# Autodesk Inventor assembly: sub assembly 2iam
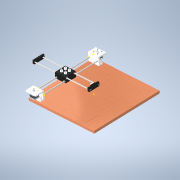
[picture p0: Inventor's stored thumbnail of the model, 180x180]
Saved by Autodesk Inventor 2021 (Build 250183000, 183)
## iProperties
Created: 2021-07-13
Part Number: sub assembly 2iam
Document SubType Name: Assembly
Designer: Michael Swaminathan
Author: Michael Swaminathan
## Documents named in this file (9)
- F:\Pattern Drawing Bot\Xy plotter Drawing Machine\sub assembly 2iam.iam
- F:\Pattern Drawing Bot\Xy plotter Drawing Machine\base.ipt
- F:\Pattern Drawing Bot\Xy plotter Drawing Machine\Motor With Support Assembly.iam
- F:\Pattern Drawing Bot\Xy plotter Drawing Machine\Guidance Rods 2.ipt
- F:\Pattern Drawing Bot\Xy plotter Drawing Machine\Central Portion Assembly.iam
- F:\Pattern Drawing Bot\Xy plotter Drawing Machine\Y-Axis.ipt
- F:\Pattern Drawing Bot\Xy plotter Drawing Machine\Y-axis on Holder.ipt
- F:\Pattern Drawing Bot\Xy plotter Drawing Machine\Rollers(2).ipt
- F:\Pattern Drawing Bot\Xy plotter Drawing Machine\roller support on y axis.ipt
## Components (12 placed, 8 different names)
1. base:1 — Rotational:2, Rotational:3
2. Motor With Support Assembly:1 [sub-assembly] — Rotational:2, Rigid:2, Rigid:3
3. Motor With Support Assembly:2 [sub-assembly] — Rotational:3, Mate:3, Mate:4
4. Guidance Rods 2:1 — Rigid:3, Mate:1, Mate:4
5. Guidance Rods 2:2 — Rigid:2, Insert:1, Mate:3
6. Central Portion Assembly:1 [sub-assembly] — Insert:1, Mate:1, Insert:2, Mate:5
7. Guidance Rods 2:3 — Mate:5, Insert:6, Mate:8
8. Guidance Rods 2:4 — Insert:2, Insert:5, Insert:12
9. Y-Axis:1 — Insert:12, Mate:8
10. Y-axis on Holder:1 — Insert:5, Insert:6, Insert:10
11. Rollers(2):1 — Insert:11
12. roller support on y axis:1 — Insert:10, Insert:11
## Relationships (16: Insert 7, Mate 5, RevoluteJoint 2, WeldJoint 2)
- Rotational:2 [RevoluteJoint]: base:1 ↔ Motor With Support Assembly:1
- Rotational:3 [RevoluteJoint]: base:1 ↔ Motor With Support Assembly:2
- Rigid:2 [WeldJoint] (-6 mm): Motor With Support Assembly:1 ↔ Guidance Rods 2:2
- Rigid:3 [WeldJoint] (-4 mm): Motor With Support Assembly:1 ↔ Guidance Rods 2:1
- Insert:1 (-250 mm): Guidance Rods 2:2 ↔ Central Portion Assembly:1
- Mate:1: Guidance Rods 2:1 ↔ Central Portion Assembly:1
- Insert:2 (260 mm): Central Portion Assembly:1 ↔ Guidance Rods 2:4
- Mate:3: Motor With Support Assembly:2 ↔ Guidance Rods 2:2
- Mate:4: Motor With Support Assembly:2 ↔ Guidance Rods 2:1
- Mate:5: Central Portion Assembly:1 ↔ Guidance Rods 2:3
- Insert:5 (-10 mm): Guidance Rods 2:4 ↔ Y-axis on Holder:1
- Insert:6 (-10 mm): Guidance Rods 2:3 ↔ Y-axis on Holder:1
- Insert:10 (7 mm): Y-axis on Holder:1 ↔ roller support on y axis:1
- Insert:11 (1 mm): Rollers(2):1 ↔ roller support on y axis:1
- Insert:12: Guidance Rods 2:4 ↔ Y-Axis:1
- Mate:8: Guidance Rods 2:3 ↔ Y-Axis:1
